# Autodesk Inventor assembly: MotorLeft
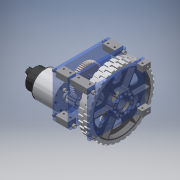
[picture p0: Inventor's stored thumbnail of the model, 180x180]
Saved by Autodesk Inventor 2019 (Build 230136000, 136)
## iProperties
Created: 2020-02-28
Part Number: MotorLeft
Document SubType Name: Assembly
Designer: james
Author: james
## Documents named in this file (15)
- F:\JimsRobot\FIRSTRobots\Design\TornadoPlatypus\MotorLeft.iam
- F:\JimsRobot\FIRSTRobots\Design\TornadoPlatypus\InsideMotorPlate.ipt
- F:\JimsRobot\FIRSTRobots\Design\Library\CTR\Falcon\217-6515 20191025.iam
- F:\JimsRobot\FIRSTRobots\Design\Library\AndyMark\FR6ZZ Bearing.ipt
- F:\JimsRobot\FIRSTRobots\Design\TornadoPlatypus\MotorSpacerBlock.ipt
- F:\JimsRobot\FIRSTRobots\Design\Library\AndyMark\Toughbox d07.ipt
- F:\JimsRobot\FIRSTRobots\Design\Library\AndyMark\6 HiGrip Asm Rev II.iam
- F:\JimsRobot\FIRSTRobots\Design\TornadoPlatypus\MotorSpacerBlock2.ipt
- F:\JimsRobot\FIRSTRobots\Design\TornadoPlatypus\MotorSpacerBlock3.ipt
- F:\JimsRobot\FIRSTRobots\Design\Library\CTR\10T_20DP_FALCON.ipt
- F:\JimsRobot\FIRSTRobots\Design\Library\Fasteners\Size-10-32\HexCap-1.ipt
- F:\JimsRobot\FIRSTRobots\Design\Library\AndyMark\am-0149 50T 20dp 375hex REV2.ipt
- F:\JimsRobot\FIRSTRobots\Design\Library\AndyMark\am-0747 16t 20dp 375h with teeth.ipt
- F:\JimsRobot\FIRSTRobots\Design\Library\AndyMark\am-0184 48T 500in Hex Bore Gear REV2 (1).ipt
- F:\JimsRobot\FIRSTRobots\Design\Library\Fasteners\Size-10-32\HexCap - .5.ipt
## Components (32 placed, 14 different names)
1. InsideMotorPlate:1 — Mate:1, Mate:2, Mate:3, Mate:5, Mate:6, Mate:8, Mate:9, Mate:10, Mate:11, Flush:1, Mate:13, Flush:3, Mate:14, Flush:4, Mate:21, Mate:22, Mate:42, Mate:44, Mate:45, Mate:46, Mate:50, Mate:59, Mate:60, Flush:11, Mate:62, Mate:63, Mate:64, Mate:65, Mate:66, Mate:67, Mate:68, Mate:69
2. 217-6515 20191025:1 [sub-assembly] — Mate:1, Mate:2, Mate:3, Mate:43
3. FR6ZZ Bearing:1 — Mate:5, Mate:6, Mate:15, Flush:5, Mate:48
4. MotorSpacerBlock:1 — Mate:9, Mate:13, Flush:3, Mate:26, Mate:28
5. MotorSpacerBlock:3 — Mate:10, Mate:11, Flush:1
6. MotorSpacerBlock:4 — Mate:8, Mate:14, Flush:4, Mate:27
7. Toughbox d07:1 — Mate:15, Flush:5, Mate:49, Mate:52
8. FR6ZZ Bearing:2 — Mate:21, Mate:22, Mate:54
9. InsideMotorPlate:2 — Mate:26, Mate:27, Mate:28, Mate:29, Mate:30, Mate:31, Mate:33, Flush:6, Mate:57, Mate:72, Mate:73, Mate:76, Mate:77
10. 6 HiGrip Asm Rev II:1 [sub-assembly] — Mate:29, Mate:30
11. MotorSpacerBlock2:2 — Mate:31, Mate:33, Flush:6, Mate:36, Mate:58
12. InsideMotorPlate:3 — Mate:36, Mate:38, Mate:39, Flush:8, Mate:40, Mate:41, Flush:9, Mate:55, Mate:56, Flush:10, Mate:58, Mate:70, Mate:71, Mate:74, Mate:75, Mate:78, Mate:79, Mate:80, Mate:81
13. MotorSpacerBlock3:1 — Mate:38, Mate:39, Flush:8
14. MotorSpacerBlock3:2 — Mate:40, Mate:41, Flush:9, Mate:57
15. 10T_20DP_FALCON:1 — Mate:42, Mate:43
16. HexCap-1:1 — Mate:44, Mate:50
17. HexCap-1:2 — Mate:45, Mate:46
18. am-0149 50T 20dp 375hex REV2:1 — Mate:48, Mate:49, Mate:51, Mate:53
19. am-0747 16t 20dp 375h with teeth:1 — Mate:51, Mate:52
20. am-0184 48T 500in Hex Bore Gear REV2 (1):1 — Mate:53, Mate:54
21. MotorSpacerBlock3:3 — Mate:59, Mate:60, Flush:11
22. MotorSpacerBlock3:4 — Mate:55, Mate:56, Flush:10
23. HexCap - .5:2 — Mate:80, Mate:81
24. HexCap - .5:3 — Mate:72, Mate:73
25. HexCap - .5:5 — Mate:64, Mate:66
26. HexCap - .5:6 — Mate:63, Mate:67
27. HexCap - .5:7 — Mate:62, Mate:65
28. HexCap - .5:8 — Mate:68, Mate:69
29. HexCap - .5:9 — Mate:70, Mate:71
30. HexCap - .5:10 — Mate:78, Mate:79
31. HexCap - .5:11 — Mate:74, Mate:75
32. HexCap - .5:12 — Mate:76, Mate:77
## Relationships (73: Mate 64, Flush 9)
- Mate:1: InsideMotorPlate:1 ↔ 217-6515 20191025:1
- Mate:2: InsideMotorPlate:1 ↔ 217-6515 20191025:1
- Mate:3: InsideMotorPlate:1 ↔ 217-6515 20191025:1
- Mate:5: InsideMotorPlate:1 ↔ FR6ZZ Bearing:1
- Mate:6: InsideMotorPlate:1 ↔ FR6ZZ Bearing:1
- Mate:8: InsideMotorPlate:1 ↔ MotorSpacerBlock:4
- Mate:9: InsideMotorPlate:1 ↔ MotorSpacerBlock:1
- Mate:10: InsideMotorPlate:1 ↔ MotorSpacerBlock:3
- Mate:11: InsideMotorPlate:1 ↔ MotorSpacerBlock:3
- Flush:1: InsideMotorPlate:1 ↔ MotorSpacerBlock:3
- Mate:13: InsideMotorPlate:1 ↔ MotorSpacerBlock:1
- Flush:3: InsideMotorPlate:1 ↔ MotorSpacerBlock:1
- Mate:14: InsideMotorPlate:1 ↔ MotorSpacerBlock:4
- Flush:4: InsideMotorPlate:1 ↔ MotorSpacerBlock:4
- Mate:15: FR6ZZ Bearing:1 ↔ Toughbox d07:1
- Flush:5: FR6ZZ Bearing:1 ↔ Toughbox d07:1
- Mate:21: InsideMotorPlate:1 ↔ FR6ZZ Bearing:2
- Mate:22: InsideMotorPlate:1 ↔ FR6ZZ Bearing:2
- Mate:26: MotorSpacerBlock:1 ↔ InsideMotorPlate:2
- Mate:27: MotorSpacerBlock:4 ↔ InsideMotorPlate:2
- Mate:28: MotorSpacerBlock:1 ↔ InsideMotorPlate:2
- Mate:29: InsideMotorPlate:2 ↔ 6 HiGrip Asm Rev II:1
- Mate:30: InsideMotorPlate:2 ↔ 6 HiGrip Asm Rev II:1
- Mate:31: InsideMotorPlate:2 ↔ MotorSpacerBlock2:2
- Mate:33: InsideMotorPlate:2 ↔ MotorSpacerBlock2:2
- Flush:6: InsideMotorPlate:2 ↔ MotorSpacerBlock2:2
- Mate:36: MotorSpacerBlock2:2 ↔ InsideMotorPlate:3
- Mate:38: InsideMotorPlate:3 ↔ MotorSpacerBlock3:1
- Mate:39: InsideMotorPlate:3 ↔ MotorSpacerBlock3:1
- Flush:8: InsideMotorPlate:3 ↔ MotorSpacerBlock3:1
- Mate:40: InsideMotorPlate:3 ↔ MotorSpacerBlock3:2
- Mate:41: InsideMotorPlate:3 ↔ MotorSpacerBlock3:2
- Flush:9: InsideMotorPlate:3 ↔ MotorSpacerBlock3:2
- Mate:42: InsideMotorPlate:1 ↔ 10T_20DP_FALCON:1
- Mate:43: 217-6515 20191025:1 ↔ 10T_20DP_FALCON:1
- Mate:44: InsideMotorPlate:1 ↔ HexCap-1:1
- Mate:45: InsideMotorPlate:1 ↔ HexCap-1:2
- Mate:46: InsideMotorPlate:1 ↔ HexCap-1:2
- Mate:48: FR6ZZ Bearing:1 ↔ am-0149 50T 20dp 375hex REV2:1
- Mate:49: Toughbox d07:1 ↔ am-0149 50T 20dp 375hex REV2:1
- Mate:50: InsideMotorPlate:1 ↔ HexCap-1:1
- Mate:51: am-0149 50T 20dp 375hex REV2:1 ↔ am-0747 16t 20dp 375h with teeth:1
- Mate:52: Toughbox d07:1 ↔ am-0747 16t 20dp 375h with teeth:1
- Mate:53: am-0149 50T 20dp 375hex REV2:1 ↔ am-0184 48T 500in Hex Bore Gear REV2 (1):1
- Mate:54: FR6ZZ Bearing:2 ↔ am-0184 48T 500in Hex Bore Gear REV2 (1):1
- Mate:55: InsideMotorPlate:3 ↔ MotorSpacerBlock3:4
- Mate:56: InsideMotorPlate:3 ↔ MotorSpacerBlock3:4
- Mate:57: InsideMotorPlate:2 ↔ MotorSpacerBlock3:2
- Flush:10: InsideMotorPlate:3 ↔ MotorSpacerBlock3:4
- Mate:58: MotorSpacerBlock2:2 ↔ InsideMotorPlate:3
- Mate:59: InsideMotorPlate:1 ↔ MotorSpacerBlock3:3
- Mate:60: InsideMotorPlate:1 ↔ MotorSpacerBlock3:3
- Flush:11: InsideMotorPlate:1 ↔ MotorSpacerBlock3:3
- Mate:62: InsideMotorPlate:1 ↔ HexCap - .5:7
- Mate:63: InsideMotorPlate:1 ↔ HexCap - .5:6
- Mate:64: InsideMotorPlate:1 ↔ HexCap - .5:5
- Mate:65: InsideMotorPlate:1 ↔ HexCap - .5:7
- Mate:66: InsideMotorPlate:1 ↔ HexCap - .5:5
- Mate:67: InsideMotorPlate:1 ↔ HexCap - .5:6
- Mate:68: InsideMotorPlate:1 ↔ HexCap - .5:8
- Mate:69: InsideMotorPlate:1 ↔ HexCap - .5:8
- Mate:70: InsideMotorPlate:3 ↔ HexCap - .5:9
- Mate:71: InsideMotorPlate:3 ↔ HexCap - .5:9
- Mate:72: InsideMotorPlate:2 ↔ HexCap - .5:3
- Mate:73: InsideMotorPlate:2 ↔ HexCap - .5:3
- Mate:74: InsideMotorPlate:3 ↔ HexCap - .5:11
- Mate:75: InsideMotorPlate:3 ↔ HexCap - .5:11
- Mate:76: InsideMotorPlate:2 ↔ HexCap - .5:12
- Mate:77: InsideMotorPlate:2 ↔ HexCap - .5:12
- Mate:78: InsideMotorPlate:3 ↔ HexCap - .5:10
- Mate:79: InsideMotorPlate:3 ↔ HexCap - .5:10
- Mate:80: InsideMotorPlate:3 ↔ HexCap - .5:2
- Mate:81: InsideMotorPlate:3 ↔ HexCap - .5:2
